# Autodesk Inventor assembly: Förderband
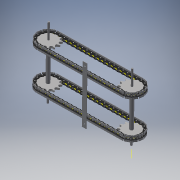
[picture p0: Inventor's stored thumbnail of the model, 180x180]
Saved by Autodesk Inventor 2018 (Build 220112000, 112)
## iProperties
Created: 2018-01-11
Part Number: Förderband
Material: Generisch
Document SubType Name: Assembly
Designer: Dominik
Author: Dominik
## Documents named in this file (6)
- C:\Users\Julian\Desktop\Schule\5AHME\Diplomarbeit\Git\fuettr_prototype\Mechanical\Inventorskizzen\Förderband.iam
- C:\Users\Julian\Desktop\Schule\5AHME\Diplomarbeit\Git\fuettr_prototype\Mechanical\Inventorskizzen\Kettenradzusammensetzung_rechts.iam
- C:\Users\Julian\Desktop\Schule\5AHME\Diplomarbeit\Git\fuettr_prototype\Mechanical\Inventorskizzen\Kettenradzusammensetzung_links.iam
- C:\Users\Julian\Desktop\Schule\5AHME\Diplomarbeit\Git\fuettr_prototype\Mechanical\Inventorskizzen\Förderbandwelle_vorne.ipt
- C:\Users\Julian\Desktop\Schule\5AHME\Diplomarbeit\Git\fuettr_prototype\Mechanical\Inventorskizzen\Förderbandwelle_hinten.ipt
- C:\Users\Julian\Desktop\Schule\5AHME\Diplomarbeit\Git\fuettr_prototype\Mechanical\Inventorskizzen\Platte_Kettenglied_unten.ipt
## Components (5 placed, 5 different names)
1. Kettenradzusammensetzung_rechts:1 [sub-assembly] — Passend:3, Passend:4, Passend:6, Passend:7
2. Kettenradzusammensetzung_links:1 [sub-assembly] — Passend:1, Passend:2, Passend:5, Passend:8, Passend:9, Passend:10
3. Förderbandwelle_vorne:1 — Passend:5, Passend:6, Passend:7
4. Förderbandwelle_hinten:1 — Passend:1, Passend:2, Passend:3, Passend:4
5. Platte_Kettenglied_unten:3 — Passend:8, Passend:9, Passend:10
## Relationships (10: Mate 10)
- Passend:1 [Mate]: Kettenradzusammensetzung_links:1 ↔ Förderbandwelle_hinten:1
- Passend:2 [Mate]: Kettenradzusammensetzung_links:1 ↔ Förderbandwelle_hinten:1
- Passend:3 [Mate]: Kettenradzusammensetzung_rechts:1 ↔ Förderbandwelle_hinten:1
- Passend:4 [Mate]: Kettenradzusammensetzung_rechts:1 ↔ Förderbandwelle_hinten:1
- Passend:5 [Mate]: Kettenradzusammensetzung_links:1 ↔ Förderbandwelle_vorne:1
- Passend:6 [Mate]: Kettenradzusammensetzung_rechts:1 ↔ Förderbandwelle_vorne:1
- Passend:7 [Mate]: Kettenradzusammensetzung_rechts:1 ↔ Förderbandwelle_vorne:1
- Passend:8 [Mate]: Kettenradzusammensetzung_links:1 ↔ Platte_Kettenglied_unten:3
- Passend:9 [Mate]: Kettenradzusammensetzung_links:1 ↔ Platte_Kettenglied_unten:3
- Passend:10 [Mate]: Kettenradzusammensetzung_links:1 ↔ Platte_Kettenglied_unten:3
